# Autodesk Inventor assembly: pc3t
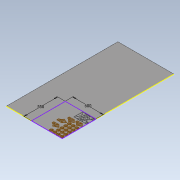
[picture p0: Inventor's stored thumbnail of the model, 180x180]
Saved by Autodesk Inventor 2020.3 (Build 243373000, 373)
## iProperties
Created: 2020-05-22
Part Number: pc3t
Document SubType Name: Assembly
Designer: aoyama
Author: aoyama
## Documents named in this file (6)
- C:\Users\aoyam\Desktop\SRDC_local\Inventor\二年機\Geminiβ\pc3t.iam
- C:\Users\aoyam\Desktop\SRDC_local\Inventor\二年機\PC板サイズ測定板.ipt
- C:\Users\aoyam\Desktop\SRDC_local\Inventor\二年機\Geminiβ\脚\ネジクランク\クランク3t.ipt
- C:\Users\aoyam\Desktop\SRDC_local\Inventor\二年機\Geminiβ\脚\脚フレーム外側後.ipt
- C:\Users\aoyam\Desktop\SRDC_local\Inventor\二年機\Geminiβ\脚\脚フレーム外側前.ipt
- C:\Users\aoyam\Desktop\SRDC_local\Inventor\二年機\Geminiβ\全体\底板.ipt
## Components (22 placed, 5 different names)
1. PC板サイズ測定板:1 — メイト:1, メイト:2, メイト:3, メイト:4, メイト:5, メイト:6, メイト:7, メイト:8, メイト:9, メイト:10, メイト:11, メイト:12, メイト:13, メイト:14, メイト:15, メイト:16, メイト:17, メイト:18, メイト:19, メイト:20, メイト:21
2. クランク3t:1 — メイト:2
3. クランク3t:2 — メイト:3
4. クランク3t:3 — メイト:5
5. クランク3t:4 — メイト:7
6. クランク3t:5 — メイト:9
7. クランク3t:6 — メイト:11
8. クランク3t:7 — メイト:14
9. クランク3t:8 — メイト:16
10. クランク3t:9 — メイト:1
11. クランク3t:10 — メイト:4
12. クランク3t:11 — メイト:6
13. クランク3t:12 — メイト:8
14. クランク3t:13 — メイト:10
15. クランク3t:14 — メイト:12
16. クランク3t:15 — メイト:13
17. クランク3t:16 — メイト:15
18. 脚フレーム外側後:1 — メイト:20
19. 脚フレーム外側前:1 — メイト:18
20. 脚フレーム外側後:2 — メイト:19
21. 脚フレーム外側前:2 — メイト:17
22. 底板:1 — メイト:21
## Relationships (21: Mate 21)
- メイト:1 [Mate]: PC板サイズ測定板:1 ↔ クランク3t:9
- メイト:2 [Mate]: PC板サイズ測定板:1 ↔ クランク3t:1
- メイト:3 [Mate]: PC板サイズ測定板:1 ↔ クランク3t:2
- メイト:4 [Mate]: PC板サイズ測定板:1 ↔ クランク3t:10
- メイト:5 [Mate]: PC板サイズ測定板:1 ↔ クランク3t:3
- メイト:6 [Mate]: PC板サイズ測定板:1 ↔ クランク3t:11
- メイト:7 [Mate]: PC板サイズ測定板:1 ↔ クランク3t:4
- メイト:8 [Mate]: PC板サイズ測定板:1 ↔ クランク3t:12
- メイト:9 [Mate]: PC板サイズ測定板:1 ↔ クランク3t:5
- メイト:10 [Mate]: PC板サイズ測定板:1 ↔ クランク3t:13
- メイト:11 [Mate]: PC板サイズ測定板:1 ↔ クランク3t:6
- メイト:12 [Mate]: PC板サイズ測定板:1 ↔ クランク3t:14
- メイト:13 [Mate]: PC板サイズ測定板:1 ↔ クランク3t:15
- メイト:14 [Mate]: PC板サイズ測定板:1 ↔ クランク3t:7
- メイト:15 [Mate]: PC板サイズ測定板:1 ↔ クランク3t:16
- メイト:16 [Mate]: PC板サイズ測定板:1 ↔ クランク3t:8
- メイト:17 [Mate]: PC板サイズ測定板:1 ↔ 脚フレーム外側前:2
- メイト:18 [Mate]: PC板サイズ測定板:1 ↔ 脚フレーム外側前:1
- メイト:19 [Mate]: PC板サイズ測定板:1 ↔ 脚フレーム外側後:2
- メイト:20 [Mate]: PC板サイズ測定板:1 ↔ 脚フレーム外側後:1
- メイト:21 [Mate]: PC板サイズ測定板:1 ↔ 底板:1
